# Autodesk Inventor assembly: Right_Lower_Engine_Mount_Assembly_V1
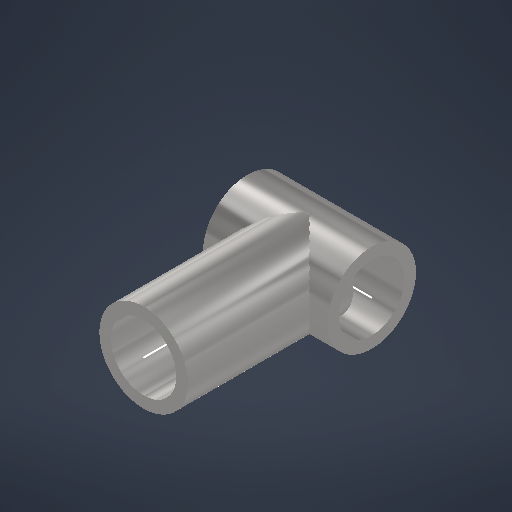
[picture p0: Inventor's stored thumbnail of the model, 512x512]
Saved by Autodesk Inventor 2026.1 (Build 301233000, 233)
## iProperties
_SolveAssemblyDoc: Frame Generator Solve Assembly
_Version: 15.0.0
Created: 2026-07-27
Part Number: Right_Lower_Engine_Mount_Assembly_V1
Document SubType Name: Assembly
Designer: share
Mass: 88.7419 g
Surface Area: 88.1235 cm^2
Volume: 11.3047 cm^3
Density: 7.85 g/cm^3
Author: share
## Documents named in this file (3)
- C:\Users\share\OneDrive\Documents\Personal Projects\GOGO Kart\CAD\GOGO_KART_FSAE\Drivetrain\Right_Lower_Engine_Mount_Assembly_V1.iam
- C:\Users\share\OneDrive\Documents\Personal Projects\GOGO Kart\CAD\GOGO_KART_FSAE\Drivetrain\Right_Upper_Engine_Mount_V1.ipt
- C:\Users\share\OneDrive\Documents\Personal Projects\GOGO Kart\CAD\GOGO_KART_FSAE\Drivetrain\Left_Engine_Mount_Assembly_V1\Right_Lower_Engine_Mount_V1_Frame.iam
## Components (2 placed, 2 different names)
1. Right_Upper_Engine_Mount_V1:1 — Flush:1, Flush:2, Flush:3
2. Right_Lower_Engine_Mount_V1_Frame:1 [sub-assembly]
## Relationships (3: Flush 3)
- Flush:1: Right_Upper_Engine_Mount_V1:1
- Flush:2: Right_Upper_Engine_Mount_V1:1
- Flush:3: Right_Upper_Engine_Mount_V1:1
